# Autodesk Inventor assembly: TZS APN 1430 inner elbow
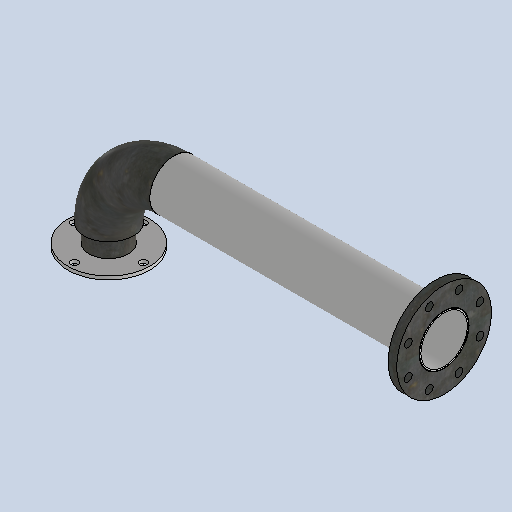
[picture p0: Inventor's stored thumbnail of the model, 512x512]
Saved by Autodesk Inventor 2025 (Build 290162010, 162A)
## iProperties
Created: 2025-07-04
Part Number: TZS APN 1430 inner elbow
Document SubType Name: Assembly
Designer: user
Author: user
## Documents named in this file (7)
- C:\Users\pokla\Documents\Inventor\TZS-Tazovskiy\TZS APN 1430 inner elbow.iam
- C:\Users\pokla\Documents\Inventor\TZS-Tazovskiy\TZS 1433 FDS tube 3.ipt
- C:\Users\pokla\Documents\Inventor\TZS-Tazovskiy\TZS 1431 FDS flange DN90.ipt
- C:\Users\pokla\Documents\Inventor\TZS-Tazovskiy\TZS 1432 FDS free flange DN90.ipt
- C:\Users\pokla\Documents\Inventor\TZS-Tazovskiy\TZS 1434 FDS tube 4.ipt
- C:\Users\pokla\Documents\Inventor\TZS-Tazovskiy\DIN 2576 Slip-On Flange for Welding Series 1 (ISO) - PN 10 80 x 88.9.ipt
- C:\Users\pokla\Documents\Inventor\TZS-Tazovskiy\JIS B 2312 90 Deg Long Elbow Steel 100A x Sch 40.ipt
## Components (6 placed, 6 different names)
1. JIS B 2312 90 Deg Long Elbow Steel 100A x Sch 40.ipt:1
2. APN 1433 FDS tube 3.ipt:1 — Rotational:1
3. APN 1434 FDS tube 4.ipt:1
4. APN 1431 FDS flange DN90.ipt:1
5. APN 1432 FDS free flange DN90.ipt:1
6. DIN 2576 Slip-On Flange for Welding Series 1 (ISO) - PN 10 80 x 88.9.ipt:1 — Rotational:1
## Relationships (5: WeldJoint 4, RevoluteJoint 1)
- [WeldJoint]: JIS B 2312 90 Deg Long Elbow Steel 100A x Sch 40.ipt:1 ↔ APN 1433 FDS tube 3.ipt:1
- [WeldJoint]: JIS B 2312 90 Deg Long Elbow Steel 100A x Sch 40.ipt:1 ↔ APN 1434 FDS tube 4.ipt:1
- [WeldJoint]: APN 1434 FDS tube 4.ipt:1 ↔ APN 1432 FDS free flange DN90.ipt:1
- [WeldJoint]: APN 1431 FDS flange DN90.ipt:1 ↔ APN 1432 FDS free flange DN90.ipt:1
- Rotational:1 [RevoluteJoint]: APN 1433 FDS tube 3.ipt:1 ↔ DIN 2576 Slip-On Flange for Welding Series 1 (ISO) - PN 10 80 x 88.9.ipt:1
